# Autodesk Inventor assembly: HbHand_MIR
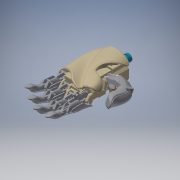
[picture p0: Inventor's stored thumbnail of the model, 180x180]
Saved by Autodesk Inventor 2017 (Build 210142000, 142)
## iProperties
Part Number: HbHand_MIR
Material: 一般
Document SubType Name: Assembly
Designer: sktom
Author: sktom
## Documents named in this file (15)
- D:\OneDrive\CAD\MAJ\hackberry\HACKberry-hardware\3D_69%inlength\Inventor_right\HbHandForChild\HbHand_MIR.iam
- D:\OneDrive\CAD\MAJ\hackberry\HACKberry-hardware\3D_69%inlength\Inventor_right\HbHandForChild\HbPalmBase03ForChild_MIR.ipt
- D:\OneDrive\CAD\MAJ\hackberry\HACKberry-hardware\3D_69%inlength\Inventor_right\HbHandForChild\bearing_683_MIR.ipt
- D:\OneDrive\CAD\MAJ\hackberry\HACKberry-hardware\3D_69%inlength\Inventor_right\HbHandForChild\HbthumbU02ForChild\HbthumbU02ForChild_MIR.iam
- D:\OneDrive\CAD\MAJ\hackberry\HACKberry-hardware\3D_69%inlength\Inventor_right\HbHandForChild\HbServoHK282A\Servo_HK282A_Hone_MIR.ipt
- D:\OneDrive\CAD\MAJ\hackberry\HACKberry-hardware\3D_69%inlength\Inventor_right\HbHandForChild\HbIndexFinger01ForChild\HbIndexFinger01ForChild_MIR.iam
- D:\OneDrive\CAD\MAJ\hackberry\HACKberry-hardware\3D_69%inlength\Inventor_right\HbHandForChild\HbFinger01ForChild\HbFinger01ForChild_MIR.iam
- D:\OneDrive\CAD\MAJ\hackberry\HACKberry-hardware\3D_69%inlength\Inventor_right\HbHandForChild\HbRing-LittleCouplerLink01ForChild_MIR.ipt
- D:\OneDrive\CAD\MAJ\hackberry\HACKberry-hardware\3D_69%inlength\Inventor_right\HbHandForChild\HbMiddle-RingCouplerLink01ForChild_MIR.ipt
- D:\OneDrive\CAD\MAJ\hackberry\HACKberry-hardware\3D_69%inlength\Inventor_right\HbHandForChild\servo\Tower Pro 9g Micro Servo SG90_MIR.iam
- D:\OneDrive\CAD\MAJ\hackberry\HACKberry-hardware\3D_69%inlength\Inventor_right\HbHandForChild\DummyASV-15MG_MIR.ipt
- D:\OneDrive\CAD\MAJ\hackberry\HACKberry-hardware\3D_69%inlength\Inventor_right\HbHandForChild\HbWristMount01ForChild_MIR.ipt
- D:\OneDrive\CAD\MAJ\hackberry\HACKberry-hardware\3D_69%inlength\Inventor_right\HbHandForChild\HbFingerMainCouplerLink01ForChild_MIR.ipt
- D:\OneDrive\CAD\MAJ\hackberry\HACKberry-hardware\3D_69%inlength\Inventor_right\HbHandForChild\DummyASV-15MGSingleHorn01_MIR.ipt
- D:\OneDrive\CAD\MAJ\hackberry\HACKberry-hardware\3D_69%inlength\Inventor_right\HbHandForChild\HbBackCover02ForChild_MIR.ipt
## Components (16 placed, 14 different names)
1. HbPalmBase03ForChild_MIR:1 — 挿入:1, 挿入:5, 挿入:4, 挿入:6, 挿入:8, 挿入:7, 挿入:10, 挿入:9, 挿入:12, 挿入:11, 挿入:16, 挿入:15, メイト:3, メイト:2, 挿入:18, 挿入:17, 挿入:23, 挿入:22
2. bearing_683_MIR:1 — 挿入:1, 挿入:2
3. HbthumbU02ForChild_MIR:1 [sub-assembly] — 挿入:2, 挿入:3
4. Servo_HK282A_Hone_MIR:1 — 挿入:5, 挿入:4, 挿入:3
5. HbIndexFinger01ForChild_MIR:1 [sub-assembly] — 挿入:6
6. HbFinger01ForChild_MIR:1 [sub-assembly] — 挿入:8, 挿入:7, 挿入:13
7. HbFinger01ForChild_MIR:2 [sub-assembly] — 挿入:10, 挿入:9, 挿入:14, 円柱状:1
8. HbFinger01ForChild_MIR:3 [sub-assembly] — 挿入:12, 挿入:11, 挿入:19, 円柱状:2
9. HbRing-LittleCouplerLink01ForChild_MIR:1 — 挿入:14, 円柱状:2
10. HbMiddle-RingCouplerLink01ForChild_MIR:1 — 挿入:13, 円柱状:1
11. Tower Pro 9g Micro Servo SG90_MIR:1 [sub-assembly] — 挿入:16, 挿入:15
12. DummyASV-15MG_MIR:1 — メイト:3, メイト:2, 挿入:20
13. HbWristMount01ForChild_MIR:1 — 挿入:18, 挿入:17
14. HbFingerMainCouplerLink01ForChild_MIR:1 — 挿入:19, 挿入:21
15. DummyASV-15MGSingleHorn01_MIR:1 — 挿入:21, 挿入:20
16. HbBackCover02ForChild_MIR:1 — 挿入:23, 挿入:22
## Relationships (27: Insert 23, Mate 2, CylindricalJoint 2)
- 挿入:1 [Insert]: HbPalmBase03ForChild_MIR:1 ↔ bearing_683_MIR:1
- 挿入:2 [Insert]: bearing_683_MIR:1 ↔ HbthumbU02ForChild_MIR:1
- 挿入:5 [Insert]: HbPalmBase03ForChild_MIR:1 ↔ Servo_HK282A_Hone_MIR:1
- 挿入:4 [Insert]: HbPalmBase03ForChild_MIR:1 ↔ Servo_HK282A_Hone_MIR:1
- 挿入:3 [Insert]: HbthumbU02ForChild_MIR:1 ↔ Servo_HK282A_Hone_MIR:1
- 挿入:6 [Insert]: HbPalmBase03ForChild_MIR:1 ↔ HbIndexFinger01ForChild_MIR:1
- 挿入:8 [Insert]: HbPalmBase03ForChild_MIR:1 ↔ HbFinger01ForChild_MIR:1
- 挿入:7 [Insert]: HbPalmBase03ForChild_MIR:1 ↔ HbFinger01ForChild_MIR:1
- 挿入:10 [Insert]: HbPalmBase03ForChild_MIR:1 ↔ HbFinger01ForChild_MIR:2
- 挿入:9 [Insert]: HbPalmBase03ForChild_MIR:1 ↔ HbFinger01ForChild_MIR:2
- 挿入:12 [Insert]: HbPalmBase03ForChild_MIR:1 ↔ HbFinger01ForChild_MIR:3
- 挿入:11 [Insert]: HbPalmBase03ForChild_MIR:1 ↔ HbFinger01ForChild_MIR:3
- 挿入:14 [Insert]: HbFinger01ForChild_MIR:2 ↔ HbRing-LittleCouplerLink01ForChild_MIR:1
- 挿入:13 [Insert]: HbFinger01ForChild_MIR:1 ↔ HbMiddle-RingCouplerLink01ForChild_MIR:1
- 挿入:16 [Insert]: HbPalmBase03ForChild_MIR:1 ↔ Tower Pro 9g Micro Servo SG90_MIR:1
- 挿入:15 [Insert]: HbPalmBase03ForChild_MIR:1 ↔ Tower Pro 9g Micro Servo SG90_MIR:1
- メイト:3 [Mate]: HbPalmBase03ForChild_MIR:1 ↔ DummyASV-15MG_MIR:1
- メイト:2 [Mate]: HbPalmBase03ForChild_MIR:1 ↔ DummyASV-15MG_MIR:1
- 挿入:18 [Insert]: HbPalmBase03ForChild_MIR:1 ↔ HbWristMount01ForChild_MIR:1
- 挿入:17 [Insert]: HbPalmBase03ForChild_MIR:1 ↔ HbWristMount01ForChild_MIR:1
- 挿入:19 [Insert] (0.1 mm): HbFinger01ForChild_MIR:3 ↔ HbFingerMainCouplerLink01ForChild_MIR:1
- 挿入:21 [Insert]: HbFingerMainCouplerLink01ForChild_MIR:1 ↔ DummyASV-15MGSingleHorn01_MIR:1
- 挿入:20 [Insert]: DummyASV-15MG_MIR:1 ↔ DummyASV-15MGSingleHorn01_MIR:1
- 挿入:23 [Insert]: HbPalmBase03ForChild_MIR:1 ↔ HbBackCover02ForChild_MIR:1
- 挿入:22 [Insert]: HbPalmBase03ForChild_MIR:1 ↔ HbBackCover02ForChild_MIR:1
- 円柱状:2 [CylindricalJoint]: HbFinger01ForChild_MIR:3 ↔ HbRing-LittleCouplerLink01ForChild_MIR:1
- 円柱状:1 [CylindricalJoint]: HbFinger01ForChild_MIR:2 ↔ HbMiddle-RingCouplerLink01ForChild_MIR:1
